# Autodesk Inventor assembly: Ensamblaje1
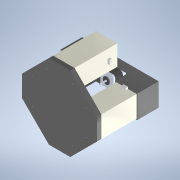
[picture p0: Inventor's stored thumbnail of the model, 180x180]
Saved by Autodesk Inventor 2021 (Build 250183000, 183)
## iProperties
Created: 2021-03-02
Part Number: Ensamblaje1
Document SubType Name: Assembly
Designer: Marc
Author: Marc
## Documents named in this file (5)
- C:\Users\Marc\Documents\Projectes\Rubik's Cube Solver\Ensamblaje1.iam
- C:\Users\Marc\Documents\Projectes\Rubik's Cube Solver\Base.ipt
- C:\Users\Marc\Documents\Projectes\Rubik's Cube Solver\Torre Motor.ipt
- C:\Users\Marc\Documents\Projectes\Rubik's Cube Solver\Nema17.ipt
- C:\Users\Marc\Documents\Projectes\Rubik's Cube Solver\Suport motor superior.ipt
## Components (12 placed, 4 different names)
1. Base:1 — Coincidencia:1, Nivelación:1, De rotación:1, Coincidencia:2, Nivelación:2, De rotación:2, Coincidencia:3, Nivelación:3, De rotación:3, Coincidencia:4, Nivelación:4, De rotación:4, Coincidencia:19
2. Torre Motor:1 — Coincidencia:3, Nivelación:3, De rotación:3, Coincidencia:5, Coincidencia:6
3. Torre Motor:2 — Coincidencia:4, Nivelación:4, De rotación:4, Coincidencia:9, Coincidencia:10
4. Torre Motor:3 — Coincidencia:1, Nivelación:1, De rotación:1, Coincidencia:7, Coincidencia:8
5. Torre Motor:4 — Coincidencia:2, Nivelación:2, De rotación:2, Coincidencia:11, Coincidencia:12, Coincidencia:13, Coincidencia:14, Coincidencia:15
6. Nema17:1 — Coincidencia:5, Coincidencia:6
7. Nema17:2 — Coincidencia:7, Coincidencia:8
8. Nema17:3 — Coincidencia:11, Coincidencia:12
9. Nema17:4 — Coincidencia:9, Coincidencia:10
10. Suport motor superior:1 — Coincidencia:13, Coincidencia:14, Coincidencia:15, Coincidencia:16, Coincidencia:17, Coincidencia:18
11. Nema17:5 — Coincidencia:16, Coincidencia:17, Coincidencia:18, Nivelación:5, Nivelación:6
12. Nema17:6 — Coincidencia:19, Nivelación:5, Nivelación:6
## Relationships (29: Mate 19, Flush 6, RevoluteJoint 4)
- Coincidencia:1 [Mate]: Base:1 ↔ Torre Motor:3
- Nivelación:1 [Flush]: Base:1 ↔ Torre Motor:3
- De rotación:1 [RevoluteJoint]: Base:1 ↔ Torre Motor:3
- Coincidencia:2 [Mate]: Base:1 ↔ Torre Motor:4
- Nivelación:2 [Flush]: Base:1 ↔ Torre Motor:4
- De rotación:2 [RevoluteJoint]: Base:1 ↔ Torre Motor:4
- Coincidencia:3 [Mate]: Base:1 ↔ Torre Motor:1
- Nivelación:3 [Flush]: Base:1 ↔ Torre Motor:1
- De rotación:3 [RevoluteJoint]: Base:1 ↔ Torre Motor:1
- Coincidencia:4 [Mate]: Base:1 ↔ Torre Motor:2
- Nivelación:4 [Flush]: Base:1 ↔ Torre Motor:2
- De rotación:4 [RevoluteJoint]: Base:1 ↔ Torre Motor:2
- Coincidencia:5 [Mate]: Torre Motor:1 ↔ Nema17:1
- Coincidencia:6 [Mate]: Torre Motor:1 ↔ Nema17:1
- Coincidencia:7 [Mate]: Torre Motor:3 ↔ Nema17:2
- Coincidencia:8 [Mate]: Torre Motor:3 ↔ Nema17:2
- Coincidencia:9 [Mate]: Torre Motor:2 ↔ Nema17:4
- Coincidencia:10 [Mate]: Torre Motor:2 ↔ Nema17:4
- Coincidencia:11 [Mate]: Torre Motor:4 ↔ Nema17:3
- Coincidencia:12 [Mate]: Torre Motor:4 ↔ Nema17:3
- Coincidencia:13 [Mate]: Torre Motor:4 ↔ Suport motor superior:1
- Coincidencia:14 [Mate] (0.5 mm): Torre Motor:4 ↔ Suport motor superior:1
- Coincidencia:15 [Mate] (0.5 mm): Torre Motor:4 ↔ Suport motor superior:1
- Coincidencia:16 [Mate]: Suport motor superior:1 ↔ Nema17:5
- Coincidencia:17 [Mate] (72.77 mm): Suport motor superior:1 ↔ Nema17:5
- Coincidencia:18 [Mate] (10.27 mm): Suport motor superior:1 ↔ Nema17:5
- Coincidencia:19 [Mate]: Base:1 ↔ Nema17:6
- Nivelación:5 [Flush]: Nema17:5 ↔ Nema17:6
- Nivelación:6 [Flush]: Nema17:5 ↔ Nema17:6
